# Autodesk Inventor assembly: Table Top and Flaps
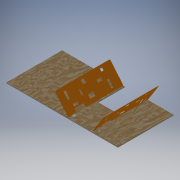
[picture p0: Inventor's stored thumbnail of the model, 180x180]
Saved by Autodesk Inventor 2016 (Build 200138000, 138)
## iProperties
Created: 2016-04-03
Part Number: Table Top and Flaps
Document SubType Name: Assembly
Designer: amycroft3
Author: amycroft3
## Documents named in this file (7)
- C:\Users\Andrea\Documents\Dropbox\Capstone CAD\Motor + Attachment\Table Top and Flaps.iam
- C:\Users\Andrea\Documents\Dropbox\Capstone CAD\Table Top .25 in.ipt
- C:\Users\Andrea\Documents\Dropbox\Capstone CAD\SideFlap.ipt
- C:\Users\Andrea\Documents\Dropbox\Capstone CAD\Hinge.iam
- C:\Users\Andrea\Documents\Dropbox\Capstone CAD\Motor + Attachment\Motor.ipt
- C:\Users\Andrea\Documents\Dropbox\Capstone CAD\Motor + Attachment\attachment.ipt
- C:\Users\Andrea\Documents\Dropbox\Capstone CAD\Motor + Attachment\Rotator.ipt
## Components (8 placed, 6 different names)
1. Table Top .25 in:1 — Mate:1, Mate:2, Mate:3, Mate:4, Mate:5, Mate:6, Mate:13, Mate:14, Mate:15
2. SideFlap:1 — Mate:10, Mate:11, Mate:12
3. SideFlap:2 — Mate:7, Mate:8, Mate:9, Mate:16
4. Hinge:1 [sub-assembly] — Mate:2, Mate:5, Mate:6, Mate:7, Mate:8, Mate:9
5. Hinge:3 [sub-assembly] — Mate:1, Mate:3, Mate:4, Mate:10, Mate:11, Mate:12
6. Motor:1 — Insert:1, Insert:2
7. attachment:1 — Insert:1, Mate:13, Mate:14, Mate:15
8. Rotator:1 — Insert:2, Mate:16
## Relationships (18: Mate 16, Insert 2)
- Mate:1: Table Top .25 in:1 ↔ Hinge:3
- Mate:2: Table Top .25 in:1 ↔ Hinge:1
- Mate:3: Table Top .25 in:1 ↔ Hinge:3
- Mate:4: Table Top .25 in:1 ↔ Hinge:3
- Mate:5: Table Top .25 in:1 ↔ Hinge:1
- Mate:6: Table Top .25 in:1 ↔ Hinge:1
- Mate:7: SideFlap:2 ↔ Hinge:1
- Mate:8: SideFlap:2 ↔ Hinge:1
- Mate:9: SideFlap:2 ↔ Hinge:1
- Mate:10: SideFlap:1 ↔ Hinge:3
- Mate:11: SideFlap:1 ↔ Hinge:3
- Mate:12: SideFlap:1 ↔ Hinge:3
- Insert:1: Motor:1 ↔ attachment:1
- Insert:2: Motor:1 ↔ Rotator:1
- Mate:13: Table Top .25 in:1 ↔ attachment:1
- Mate:14: Table Top .25 in:1 ↔ attachment:1
- Mate:15: Table Top .25 in:1 ↔ attachment:1
- Mate:16: SideFlap:2 ↔ Rotator:1
